# Autodesk Inventor assembly: masterswitchfinal
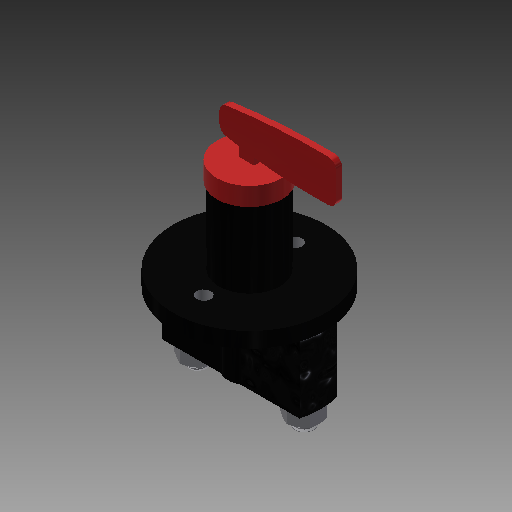
[picture p0: Inventor's stored thumbnail of the model, 512x512]
Saved by Autodesk Inventor 2019 (Build 230136000, 136)
## iProperties
Created: 2020-02-15
Part Number: masterswitchfinal
Document SubType Name: Assembly
Designer: brosemej
Author: brosemej
## Documents named in this file (4)
- G:\Shared drives\FSAE EV\FSAE EV 2020-2021\Subsystem Folders\Interconnect\MRESET.iam
- G:\Shared drives\FSAE EV\FSAE EV 2020-2021\Subsystem Folders\Interconnect\masterswitch.ipt
- G:\Shared drives\FSAE EV\FSAE EV 2020-2021\Subsystem Folders\Interconnect\m8 nut hex.ipt
- G:\Shared drives\FSAE EV\FSAE EV 2020-2021\Subsystem Folders\Interconnect\SCREW M8X1.25 stud.ipt
## Components (5 placed, 3 different names)
1. masterswitch:1 — Mate:1, Mate:2, Mate:3, Mate:4
2. m8 nut hex:1 — Mate:1
3. m8 nut hex:2 — Mate:2
4. SCREW M8X1.25 stud:1 — Mate:3
5. SCREW M8X1.25 stud:2 — Mate:4
## Relationships (4: Mate 4)
- Mate:1: masterswitch:1 ↔ m8 nut hex:1
- Mate:2: masterswitch:1 ↔ m8 nut hex:2
- Mate:3: masterswitch:1 ↔ SCREW M8X1.25 stud:1
- Mate:4: masterswitch:1 ↔ SCREW M8X1.25 stud:2
